# Autodesk Inventor assembly: steering_hub_assembly_right
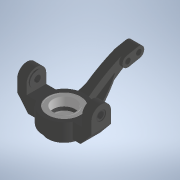
[picture p0: Inventor's stored thumbnail of the model, 180x180]
Saved by Autodesk Inventor 2020 (Build 240168000, 168)
## iProperties
Created: 2019-12-09
Part Number: steering_hub_assembly_right
Document SubType Name: Assembly
Designer: maste
Author: maste
## Documents named in this file (5)
- C:\Users\maste\Documents\GitHub\autobot\robot_model\steering_hub_assembly_right.iam
- C:\Users\maste\Documents\GitHub\autobot\robot_model\RCT-P006_steering_knuckle_right_OK.ipt
- C:\Users\maste\Documents\GitHub\autobot\robot_model\B6700ZZ.ipt
- C:\Users\maste\Documents\GitHub\autobot\robot_model\BR115ZZ.ipt
- C:\Users\maste\Documents\GitHub\autobot\robot_model\RCT-H019.ipt
## Components (5 placed, 4 different names)
1. RCT-P006_steering_knuckle_right_OK:1 — Mate:1, Mate:2, Mate:3, Mate:4, Mate:5, Mate:6, Mate:7, Mate:8
2. B6700ZZ:1 — Mate:1, Mate:2
3. BR115ZZ:1 — Mate:3, Mate:4
4. RCT-H019:1 — Mate:5, Mate:6
5. RCT-H019:2 — Mate:7, Mate:8
## Relationships (8: Mate 8)
- Mate:1: RCT-P006_steering_knuckle_right_OK:1 ↔ B6700ZZ:1
- Mate:2: RCT-P006_steering_knuckle_right_OK:1 ↔ B6700ZZ:1
- Mate:3: RCT-P006_steering_knuckle_right_OK:1 ↔ BR115ZZ:1
- Mate:4: RCT-P006_steering_knuckle_right_OK:1 ↔ BR115ZZ:1
- Mate:5: RCT-P006_steering_knuckle_right_OK:1 ↔ RCT-H019:1
- Mate:6: RCT-P006_steering_knuckle_right_OK:1 ↔ RCT-H019:1
- Mate:7: RCT-P006_steering_knuckle_right_OK:1 ↔ RCT-H019:2
- Mate:8: RCT-P006_steering_knuckle_right_OK:1 ↔ RCT-H019:2
